# Autodesk Inventor assembly: Base_Plate_Assembly
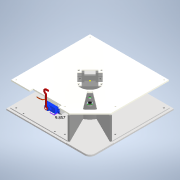
[picture p0: Inventor's stored thumbnail of the model, 180x180]
Saved by Autodesk Inventor 2022 (Build 260153000, 153)
## iProperties
Created: 2023-02-28
Part Number: Base_Plate_Assembly
Document SubType Name: Assembly
Designer: zarek
Author: zarek
## Documents named in this file (8)
- C:\Users\zarek\OneDrive\Desktop\Random New Stuff\SPB\Inside Mechanisms.iam
- C:\Users\zarek\OneDrive\Desktop\Random New Stuff\SPB\GrabCad Parts\Pi camera module3 (1).ipt
- C:\Users\zarek\OneDrive\Desktop\Random New Stuff\SPB\Motor_Holder.ipt
- C:\Users\zarek\OneDrive\Desktop\Random New Stuff\SPB\Camera_Holder.ipt
- C:\Users\zarek\OneDrive\Desktop\Random New Stuff\SPB\Drop_Plate - Copy.ipt
- C:\Users\zarek\OneDrive\Desktop\Random New Stuff\SPB\Servo&Holder.iam
- C:\Users\zarek\OneDrive\Desktop\Random New Stuff\SPB\Hook.ipt
- C:\Users\zarek\OneDrive\Desktop\Random New Stuff\SPB\Base_Plate_2_Solo_Up.ipt
## Components (7 placed, 7 different names)
1. Motor_Holder:1 — Rotational:2, Rigid:3
2. Pi camera module3 (1):1 — Rotational:1
3. Camera_Holder:1 — Rotational:1
4. Drop_Plate - Copy:1 — Rotational:2, Rotational:3
5. Servo&Holder:1 [sub-assembly] — Rotational:3, Rigid:2
6. Hook:1 — Rigid:2
7. Base_Plate_2_Solo_Up:1 — Rigid:3
## Relationships (5: RevoluteJoint 3, WeldJoint 2)
- Rotational:1 [RevoluteJoint]: Pi camera module3 (1):1 ↔ Camera_Holder:1
- Rotational:2 [RevoluteJoint]: Motor_Holder:1 ↔ Drop_Plate - Copy:1
- Rotational:3 [RevoluteJoint]: Drop_Plate - Copy:1 ↔ Servo&Holder:1
- Rigid:2 [WeldJoint]: Servo&Holder:1 ↔ Hook:1
- Rigid:3 [WeldJoint]: Motor_Holder:1 ↔ Base_Plate_2_Solo_Up:1
